# Autodesk Inventor assembly: xy ubis mount arm
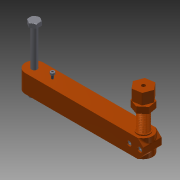
[picture p0: Inventor's stored thumbnail of the model, 180x180]
Saved by Autodesk Inventor 2013 (Build 170138000, 138)
## iProperties
Created: 2013-10-15
Part Number: xy ubis mount arm
Document SubType Name: Assembly
Designer: employee
Author: employee
## Documents named in this file (12)
- C:\Users\employee\Desktop\new wally\xy ubis mount arm.iam
- C:\Users\employee\Desktop\new wally\xy ubis mount arm.ipt
- C:\Users\employee\Desktop\new wally\m3 nut.ipt
- C:\Users\employee\Desktop\new wally\M3x20.ipt
- C:\Users\employee\Desktop\new wally\M3x16.ipt
- C:\Users\employee\Desktop\new wally\M8 nut.ipt
- C:\Users\employee\Desktop\new wally\M8x85.ipt
- C:\Users\employee\Desktop\new wally\bowden nut.ipt
- C:\Users\employee\Desktop\new wally\lock nut.ipt
- C:\Users\employee\Desktop\new wally\hub screw.ipt
- C:\Users\employee\Desktop\new wally\hub washer.ipt
- C:\Users\employee\Desktop\new wally\m4 nut.ipt
## Components (13 placed, 11 different names)
1. xy ubis mount arm:1 — Angle:1, Angle:2, Insert:2, Insert:3, Insert:5, Insert:6, Insert:7, Insert:8, Insert:9, Mate:1, Mate:2, Insert:10, Insert:11
2. Hex Nut Metric M3 x 0.5:2 — Angle:2, Insert:3
3. Hex Nut Metric M3 x 0.5:3 — Angle:1, Insert:2
4. Forged Socket Head Cap Screw - Metric M3x0.5 x 20:1 — Insert:5
5. Forged Socket Head Cap Screw - Metric M3x0.5 x 20:2 — Insert:6
6. Forged Socket Head Cap Screw - Metric M3x0.5 x 16:1 — Insert:7
7. Hex Nut Metric M8 x 1.25:1 — Insert:9
8. Hex Bolt - Metric M8 x 1.25 x 70:1 — Insert:8
9. bowden nut:1 — Mate:3, Mate:4
10. lock nut:1 — Mate:1, Mate:2, Mate:3
11. hub screw:1 — Insert:10, Mate:4, Angle:4, Insert:12
12. hub washer:1 — Insert:11
13. m4 nut:1 — Angle:4, Insert:12
## Relationships (17: Insert 10, Mate 4, Angle 3)
- Angle:1 (0 deg): xy ubis mount arm:1 ↔ Hex Nut Metric M3 x 0.5:3
- Angle:2 (0 deg): xy ubis mount arm:1 ↔ Hex Nut Metric M3 x 0.5:2
- Insert:2: xy ubis mount arm:1 ↔ Hex Nut Metric M3 x 0.5:3
- Insert:3: xy ubis mount arm:1 ↔ Hex Nut Metric M3 x 0.5:2
- Insert:5: xy ubis mount arm:1 ↔ Forged Socket Head Cap Screw - Metric M3x0.5 x 20:1
- Insert:6: xy ubis mount arm:1 ↔ Forged Socket Head Cap Screw - Metric M3x0.5 x 20:2
- Insert:7 (5 mm): xy ubis mount arm:1 ↔ Forged Socket Head Cap Screw - Metric M3x0.5 x 16:1
- Insert:8 (51.5 mm): xy ubis mount arm:1 ↔ Hex Bolt - Metric M8 x 1.25 x 70:1
- Insert:9: xy ubis mount arm:1 ↔ Hex Nut Metric M8 x 1.25:1
- Mate:1: xy ubis mount arm:1 ↔ lock nut:1
- Mate:2 (26.5 mm): xy ubis mount arm:1 ↔ lock nut:1
- Mate:3: bowden nut:1 ↔ lock nut:1
- Insert:10: xy ubis mount arm:1 ↔ hub screw:1
- Mate:4: bowden nut:1 ↔ hub screw:1
- Insert:11: xy ubis mount arm:1 ↔ hub washer:1
- Angle:4 (0 deg): hub screw:1 ↔ m4 nut:1
- Insert:12: hub screw:1 ↔ m4 nut:1
